# Autodesk Inventor assembly: Drone assembly
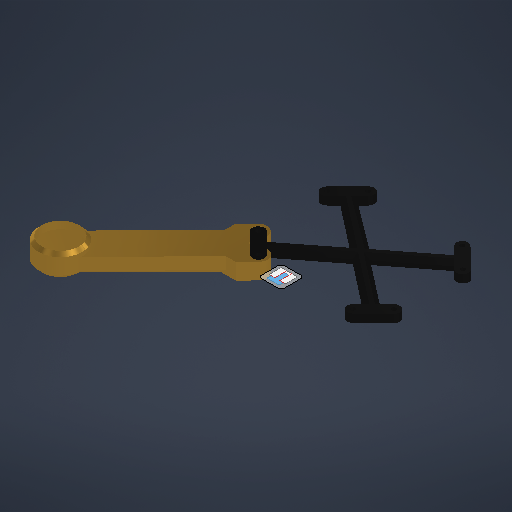
[picture p0: Inventor's stored thumbnail of the model, 512x512]
Saved by Autodesk Inventor 2026.1 (Build 301233000, 233)
## iProperties
Created: 2025-07-27
Part Number: Drone assembly
Document SubType Name: Assembly
Designer: rohit
Author: rohit
## Documents named in this file (3)
- C:\Users\rohit\OneDrive\Documents\Drone assembly.iam
- C:\Users\rohit\OneDrive\Documents\Inventor\Drone_arm.ipt
- C:\Users\rohit\OneDrive\Documents\Inventor\Drone_cross.ipt
## Components (2 placed, 2 different names)
1. Drone_arm:1 — Insert:1
2. Drone_cross:1 — Insert:1
## Relationships (1: Insert 1)
- Insert:1: Drone_arm:1 ↔ Drone_cross:1
